# Autodesk Inventor assembly: Assembly1
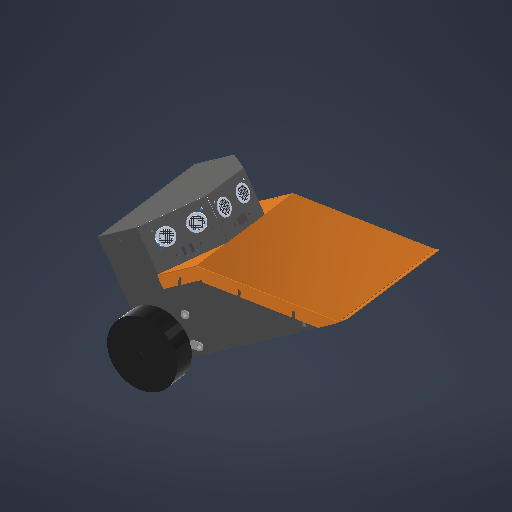
[picture p0: Inventor's stored thumbnail of the model, 512x512]
Saved by Autodesk Inventor 2026.2 (Build 302298000, 298)
## iProperties
Created: 2026-03-06
Part Number: Assembly1
Document SubType Name: Assembly
Designer: User
Author: User
## Documents named in this file (7)
- C:\Users\User\Documents\3D\robo sumo\Assembly1.iam
- C:\Users\User\Documents\3D\robo sumo\qveda_korpusi.ipt
- C:\Users\User\Documents\3D\robo sumo\5840-31ZY D8\5840-31ZY D8\5840-31ZY D8.ipt
- C:\Users\User\Documents\3D\robo sumo\kapoti.ipt
- C:\Users\User\Documents\3D\robo sumo\saxuravi.ipt
- C:\Users\User\Documents\3D\robo sumo\weel.ipt
- C:\Users\User\Documents\3D\robo sumo\HC-SR04\HC-SR04\HC-SR04.iam
## Components (10 placed, 6 different names)
1. qveda_korpusi:1 — Mate:1, Mate:2, Mate:3, Mate:4, Mate:5, Mate:6, Mate:7, Mate:8, Mate:9, Mate:10, Mate:11, Mate:12
2. 5840-31ZY D8:1 — Mate:4, Mate:5, Mate:6, Mate:15, Mate:16
3. 5840-31ZY D8:2 — Mate:1, Mate:2, Mate:3, Mate:13, Mate:14
4. kapoti:1 — Mate:7, Mate:8, Mate:9
5. saxuravi:1 — Mate:10, Mate:11, Mate:12, Insert:1, Angle:1, Insert:2, Insert:3, Angle:2, Angle:3
6. weel:1 — Mate:13, Mate:14
7. weel:2 — Mate:15, Mate:16
8. HC-SR04:1 [sub-assembly] — Insert:1, Angle:1
9. HC-SR04:2 [sub-assembly] — Insert:2, Angle:2
10. HC-SR04:3 [sub-assembly] — Insert:3, Angle:3
## Relationships (22: Mate 16, Insert 3, Angle 3)
- Mate:1: qveda_korpusi:1 ↔ 5840-31ZY D8:2
- Mate:2: qveda_korpusi:1 ↔ 5840-31ZY D8:2
- Mate:3: qveda_korpusi:1 ↔ 5840-31ZY D8:2
- Mate:4: qveda_korpusi:1 ↔ 5840-31ZY D8:1
- Mate:5: qveda_korpusi:1 ↔ 5840-31ZY D8:1
- Mate:6: qveda_korpusi:1 ↔ 5840-31ZY D8:1
- Mate:7: qveda_korpusi:1 ↔ kapoti:1
- Mate:8: qveda_korpusi:1 ↔ kapoti:1
- Mate:9: qveda_korpusi:1 ↔ kapoti:1
- Mate:10: qveda_korpusi:1 ↔ saxuravi:1
- Mate:11: qveda_korpusi:1 ↔ saxuravi:1
- Mate:12: qveda_korpusi:1 ↔ saxuravi:1
- Mate:13: 5840-31ZY D8:2 ↔ weel:1
- Mate:14: 5840-31ZY D8:2 ↔ weel:1
- Mate:15: 5840-31ZY D8:1 ↔ weel:2
- Mate:16: 5840-31ZY D8:1 ↔ weel:2
- Insert:1: saxuravi:1 ↔ HC-SR04:1
- Angle:1 (90 deg): saxuravi:1 ↔ HC-SR04:1
- Insert:2: saxuravi:1 ↔ HC-SR04:2
- Insert:3: saxuravi:1 ↔ HC-SR04:3
- Angle:2 (90 deg): saxuravi:1 ↔ HC-SR04:2
- Angle:3 (90 deg): saxuravi:1 ↔ HC-SR04:3
